# Autodesk Inventor assembly: ABD_Ankle_Version 1.0
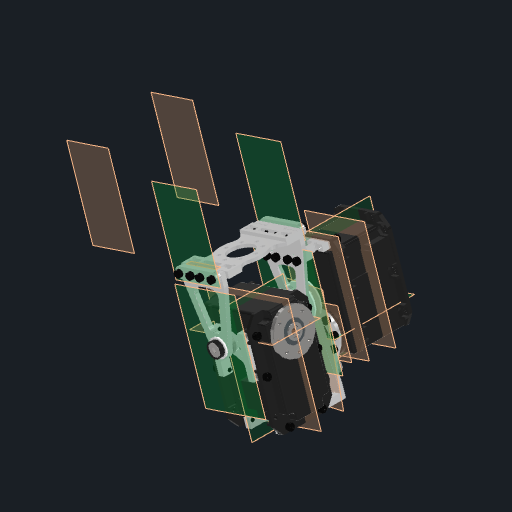
[picture p0: Inventor's stored thumbnail of the model, 512x512]
Saved by Autodesk Inventor 2024 (Build 280153000, 153)
## iProperties
Created: 2024-01-25
Part Number: ABD_Ankle_Version 1.0
Document SubType Name: Assembly
Designer: ASUS
Mass: 367.451 g
Surface Area: 648.88 cm^2
Volume: 184.634 cm^3
Author: ASUS
## Documents named in this file (21)
- C:\Users\김대겸\Desktop\2024_Robit_Hardware\ROBOCUP_2024_eindhoven\부품\Lower_Body\Anti_Backlash_Disk\ABD_Ankle_Version 1.0.iam
- C:\Users\김대겸\Desktop\2024_Robit_Hardware\ROBOCUP_2024_eindhoven\부품\ROBOTIS(Inventor 2023 ver.)\다이나믹셀\MX-106T+idle.ipt.iam
- C:\Users\김대겸\Desktop\2024_Robit_Hardware\ROBOCUP_2024_eindhoven\부품\Lower_Body\Leg\Roll_Fixation_R.ipt
- C:\Users\김대겸\Desktop\2024_Robit_Hardware\ROBOCUP_2024_eindhoven\부품\Lower_Body\Anti_Backlash_Disk\Slider_crank_horn.ipt
- C:\Users\김대겸\Desktop\2024_Robit_Hardware\ROBOCUP_2024_eindhoven\부품\Lower_Body\Leg\Roll_Fixation_L.ipt
- C:\Users\김대겸\Desktop\2024_Robit_Hardware\ROBOCUP_2024_eindhoven\부품\Lower_Body\Leg\Roll_Fixation_Frame.ipt
- C:\Users\김대겸\Desktop\2024_Robit_Hardware\ROBOCUP_2024_eindhoven\부품\Lower_Body\Anti_Backlash_Disk\Leg_joint_slider_frame.ipt
- C:\Users\김대겸\Desktop\2024_Robit_Hardware\ROBOCUP_2024_eindhoven\부품\Lower_Body\Leg\Roll_Fixation_Frame_Back.ipt
- C:\Users\김대겸\Desktop\2024_Robit_Hardware\ROBOCUP_2024_eindhoven\부품\Lower_Body\Leg\106_Slider_Fixation.ipt
- C:\Users\김대겸\Desktop\2024_Robit_Hardware\ROBOCUP_2024_eindhoven\부품\Lower_Body\Hip joint of the waist\hip joint fix washer.ipt
- C:\Users\김대겸\Desktop\2024_Robit_Hardware\ROBOCUP_2024_eindhoven\부품\Lower_Body\Leg\Roll_Fixation_Frameto64.ipt
- C:\Users\김대겸\Desktop\2024_Robit_Hardware\ROBOCUP_2024_eindhoven\부품\Lower_Body\Foot\Ankle_Footbase_Connector.ipt
- C:\Users\김대겸\Desktop\2024_Robit_Hardware\ROBOCUP_2024_eindhoven\부품\Bolt_Washer_Nut\Roll_Fixation_Frame_8mm_Set.iam
- C:\Users\김대겸\Desktop\2024_Robit_Hardware\ROBOCUP_2024_eindhoven\부품\Bolt_Washer_Nut\CSH-ST-M2_5-8_203.ipt
- C:\Users\김대겸\Desktop\2024_Robit_Hardware\ROBOCUP_2024_eindhoven\부품\Bolt_Washer_Nut\hip_joint_fix_washer_10mm_Set.iam
- C:\Users\김대겸\Desktop\2024_Robit_Hardware\ROBOCUP_2024_eindhoven\부품\Bolt_Washer_Nut\ABD_4mm_set.iam
- C:\Users\김대겸\Desktop\2024_Robit_Hardware\ROBOCUP_2024_eindhoven\부품\Bolt_Washer_Nut\ABD_STRUCTURE\Front_Frame_Fixer.iam
- C:\Users\김대겸\Desktop\2024_Robit_Hardware\ROBOCUP_2024_eindhoven\부품\Bolt_Washer_Nut\ABD_STRUCTURE\Rear_Frame_Fixer.iam
- C:\Users\김대겸\Desktop\2024_Robit_Hardware\ROBOCUP_2024_eindhoven\부품\Bolt_Washer_Nut\ABD_STRUCTURE\Crank_Slider_Fixer.iam
- C:\Users\김대겸\Desktop\2024_Robit_Hardware\ROBOCUP_2024_eindhoven\부품\ROBOTIS(Inventor 2023 ver.)\다이나믹셀\MX-64T.ipt
- MX-106T+idle.ipt
## Components (30 placed, 19 different names)
1. MX-106T+idle.ipt:1 [sub-assembly] — 삽입:8, 메이트:58, 삽입:9, 메이트:59, 삽입:10, 메이트:60
2. Roll_Fixation_R:1 — 메이트:51, 각도:1, 삽입:2
3. Slider_crank_horn:1 — 삽입:3, 삽입:19, 삽입:20, 메이트:69
4. Roll_Fixation_L:1 — 메이트:52, 각도:2, 삽입:4
5. Roll_Fixation_Frame:1 — 메이트:51, 삽입:1, 메이트:54
6. Leg_joint_slider_frame:1 — 메이트:53, 삽입:17, 삽입:18, 메이트:63, 메이트:70
7. Roll_Fixation_Frame_Back:1 — 메이트:47, 메이트:49, 메이트:50, 메이트:52, 메이트:53, 플러쉬:1, 삽입:13, 삽입:16
8. 106_Slider_Fixation:1
9. hip joint fix washer:1 — 메이트:48, 삽입:5, 메이트:55
10. hip joint fix washer:2 — 삽입:6, 메이트:56
11. Roll_Fixation_Frameto64:1 — 플러쉬:1, 삽입:14, 삽입:15, 메이트:64, 메이트:66, 메이트:68
12. Ankle_Footbase_Connector:2 — 메이트:47, 메이트:48, 메이트:49, 메이트:50, 삽입:1
13. Roll_Fixation_Frame_8mm_Set:1 [sub-assembly] — 삽입:9, 메이트:59
14. Roll_Fixation_Frame_8mm_Set:2 [sub-assembly] — 삽입:10, 메이트:60
15. CSH-ST-M2_5-8_203:1 — 삽입:18
16. CSH-ST-M2_5-8_203:2 — 삽입:17
17. Roll_Fixation_Frame_8mm_Set:3 [sub-assembly] — 삽입:8, 메이트:58
18. hip_joint_fix_washer_10mm_Set:1 [sub-assembly] — 삽입:5, 메이트:55
19. hip_joint_fix_washer_10mm_Set:2 [sub-assembly] — 삽입:6, 메이트:56
20. CSH-ST-M2_5-8_203:3 — 삽입:15
21. CSH-ST-M2_5-8_203:4 — 삽입:13
22. CSH-ST-M2_5-8_203:5 — 삽입:14
23. CSH-ST-M2_5-8_203:6 — 삽입:16
24. Front_Frame_Fixer:1 [sub-assembly] — 각도:1, 삽입:2, 메이트:54
25. Rear_Frame_Fixer:1 [sub-assembly] — 각도:2, 삽입:4
26. Crank_Slider_Fixer:1 [sub-assembly] — 삽입:3, 메이트:63, 메이트:70
27. CSH-ST-M2_5-8_203:7 — 메이트:65, 메이트:66
28. CSH-ST-M2_5-8_203:8 — 메이트:67, 메이트:68
29. MX-64T:1 — 삽입:19, 메이트:64, 메이트:65, 메이트:67
30. ABD_4mm_set:1 [sub-assembly] — 삽입:20, 메이트:69
## Relationships (64: Mate 44, Insert 17, Angle 2, Flush 1)
- [Mate] (0.05 mm): MX-106T+idle.ipt:1 ↔ Roll_Fixation_R:1
- [Mate] (0.05 mm): MX-106T+idle.ipt:1 ↔ Roll_Fixation_L:1
- [Mate]: MX-106T+idle.ipt:1 ↔ Roll_Fixation_L:1
- [Mate]: MX-106T+idle.ipt:1 ↔ Roll_Fixation_L:1
- [Mate]: MX-106T+idle.ipt:1 ↔ Roll_Fixation_L:1
- [Mate]: MX-106T+idle.ipt:1 ↔ Roll_Fixation_R:1
- [Mate]: MX-106T+idle.ipt:1 ↔ Roll_Fixation_R:1
- [Mate]: Roll_Fixation_Frame:1 ↔ Roll_Fixation_Frame_Back:1
- [Mate]: Leg_joint_slider_frame:1 ↔ 106_Slider_Fixation:1
- [Mate]: Leg_joint_slider_frame:1 ↔ 106_Slider_Fixation:1
- [Mate]: Leg_joint_slider_frame:1 ↔ 106_Slider_Fixation:1
- [Mate] (0.05 mm): MX-106T+idle.ipt:1 ↔ 106_Slider_Fixation:1
- [Mate]: MX-106T+idle.ipt:1 ↔ 106_Slider_Fixation:1
- [Mate]: MX-106T+idle.ipt:1 ↔ 106_Slider_Fixation:1
- [Mate]: MX-106T+idle.ipt:1 ↔ 106_Slider_Fixation:1
- [Mate]: Roll_Fixation_Frame:1 ↔ hip joint fix washer:1
- [Mate]: Roll_Fixation_Frame:1 ↔ hip joint fix washer:1
- [Mate]: Roll_Fixation_Frame:1 ↔ hip joint fix washer:1
- [Mate]: Roll_Fixation_Frame_Back:1 ↔ hip joint fix washer:2
- [Mate]: Roll_Fixation_Frame_Back:1 ↔ hip joint fix washer:2
- [Mate]: Roll_Fixation_Frame_Back:1 ↔ hip joint fix washer:2
- [Mate]: Roll_Fixation_Frame_Back:1 ↔ Roll_Fixation_Frameto64:1
- [Mate]: Roll_Fixation_Frame_Back:1 ↔ Roll_Fixation_Frameto64:1
- 메이트:47 [Mate]: Roll_Fixation_Frame_Back:1 ↔ Ankle_Footbase_Connector:2
- 메이트:48 [Mate]: hip joint fix washer:1 ↔ Ankle_Footbase_Connector:2
- 메이트:49 [Mate]: Roll_Fixation_Frame_Back:1 ↔ Ankle_Footbase_Connector:2
- 메이트:50 [Mate]: Roll_Fixation_Frame_Back:1 ↔ Ankle_Footbase_Connector:2
- 메이트:51 [Mate]: Roll_Fixation_R:1 ↔ Roll_Fixation_Frame:1
- 메이트:52 [Mate]: Roll_Fixation_L:1 ↔ Roll_Fixation_Frame_Back:1
- 메이트:53 [Mate]: Leg_joint_slider_frame:1 ↔ Roll_Fixation_Frame_Back:1
- 삽입:1 [Insert]: Roll_Fixation_Frame:1 ↔ Ankle_Footbase_Connector:2
- 각도:1 [Angle] (0 deg): Roll_Fixation_R:1 ↔ Front_Frame_Fixer:1
- 삽입:2 [Insert]: Roll_Fixation_R:1 ↔ Front_Frame_Fixer:1
- 삽입:3 [Insert]: Slider_crank_horn:1 ↔ Crank_Slider_Fixer:1
- 각도:2 [Angle] (0 deg): Roll_Fixation_L:1 ↔ Rear_Frame_Fixer:1
- 삽입:4 [Insert]: Roll_Fixation_L:1 ↔ Rear_Frame_Fixer:1
- 메이트:54 [Mate]: Roll_Fixation_Frame:1 ↔ Front_Frame_Fixer:1
- 삽입:5 [Insert]: hip joint fix washer:1 ↔ hip_joint_fix_washer_10mm_Set:1
- 메이트:55 [Mate]: hip joint fix washer:1 ↔ hip_joint_fix_washer_10mm_Set:1
- 삽입:6 [Insert]: hip joint fix washer:2 ↔ hip_joint_fix_washer_10mm_Set:2
- 메이트:56 [Mate]: hip joint fix washer:2 ↔ hip_joint_fix_washer_10mm_Set:2
- 삽입:8 [Insert]: MX-106T+idle.ipt:1 ↔ Roll_Fixation_Frame_8mm_Set:3
- 메이트:58 [Mate]: MX-106T+idle.ipt:1 ↔ Roll_Fixation_Frame_8mm_Set:3
- 삽입:9 [Insert]: MX-106T+idle.ipt:1 ↔ Roll_Fixation_Frame_8mm_Set:1
- 메이트:59 [Mate]: MX-106T+idle.ipt:1 ↔ Roll_Fixation_Frame_8mm_Set:1
- 삽입:10 [Insert]: MX-106T+idle.ipt:1 ↔ Roll_Fixation_Frame_8mm_Set:2
- 메이트:60 [Mate]: MX-106T+idle.ipt:1 ↔ Roll_Fixation_Frame_8mm_Set:2
- 플러쉬:1 [Flush]: Roll_Fixation_Frame_Back:1 ↔ Roll_Fixation_Frameto64:1
- 삽입:13 [Insert]: Roll_Fixation_Frame_Back:1 ↔ CSH-ST-M2_5-8_203:4
- 삽입:14 [Insert]: Roll_Fixation_Frameto64:1 ↔ CSH-ST-M2_5-8_203:5
- 삽입:15 [Insert]: Roll_Fixation_Frameto64:1 ↔ CSH-ST-M2_5-8_203:3
- 삽입:16 [Insert]: Roll_Fixation_Frame_Back:1 ↔ CSH-ST-M2_5-8_203:6
- 삽입:17 [Insert]: Leg_joint_slider_frame:1 ↔ CSH-ST-M2_5-8_203:2
- 삽입:18 [Insert]: Leg_joint_slider_frame:1 ↔ CSH-ST-M2_5-8_203:1
- 삽입:19 [Insert]: Slider_crank_horn:1 ↔ MX-64T:1
- 메이트:63 [Mate]: Leg_joint_slider_frame:1 ↔ Crank_Slider_Fixer:1
- 메이트:64 [Mate]: Roll_Fixation_Frameto64:1 ↔ MX-64T:1
- 메이트:65 [Mate]: CSH-ST-M2_5-8_203:7 ↔ MX-64T:1
- 메이트:66 [Mate]: Roll_Fixation_Frameto64:1 ↔ CSH-ST-M2_5-8_203:7
- 메이트:67 [Mate]: CSH-ST-M2_5-8_203:8 ↔ MX-64T:1
- 메이트:68 [Mate]: Roll_Fixation_Frameto64:1 ↔ CSH-ST-M2_5-8_203:8
- 삽입:20 [Insert]: Slider_crank_horn:1 ↔ ABD_4mm_set:1
- 메이트:69 [Mate]: Slider_crank_horn:1 ↔ ABD_4mm_set:1
- 메이트:70 [Mate]: Leg_joint_slider_frame:1 ↔ Crank_Slider_Fixer:1
